# Autodesk Inventor assembly: ShfiterAssy
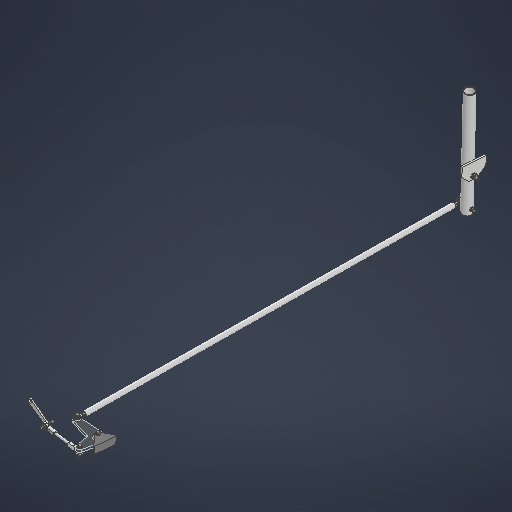
[picture p0: Inventor's stored thumbnail of the model, 512x512]
Saved by Autodesk Inventor 2026.2 (Build 302298010, 298A)
## iProperties
Created: 2026-07-07
Part Number: ShfiterAssy
Document SubType Name: Assembly
Designer: tasle
Author: tasle
## Documents named in this file (18)
- C:\Users\tasle\Documents\PersonalProjects\FSAE\GOGO_FSAE_CAD\Shifter\ShfiterAssy.iam
- C:\Users\tasle\Documents\PersonalProjects\FSAE\GOGO_FSAE_CAD\Shifter\crank.ipt
- C:\Users\tasle\Documents\PersonalProjects\FSAE\GOGO_FSAE_CAD\Shifter\59935K71_Ball Joint Rod End\59935K71_Ball Joint Rod End\59935K71_Ball Joint Rod End.ipt
- C:\Users\tasle\Documents\PersonalProjects\FSAE\GOGO_FSAE_CAD\Shifter\threadedtubeshort.ipt
- C:\Users\tasle\Documents\Inventor\Content Center Files\R2026\en-US\ISO 4162\ISO 4162 - M5 x 25.ipt
- C:\Users\tasle\Documents\Inventor\Content Center Files\R2026\en-US\ISO 4161\ISO 4161 - M5(1).ipt
- C:\Users\tasle\Documents\PersonalProjects\FSAE\GOGO_FSAE_CAD\Shifter\ShifterBracket.ipt
- C:\Users\tasle\Documents\PersonalProjects\FSAE\GOGO_FSAE_CAD\Shifter\BellCrank.ipt
- C:\Users\tasle\Documents\PersonalProjects\FSAE\GOGO_FSAE_CAD\Shifter\Bearing.ipt
- C:\Users\tasle\Documents\PersonalProjects\FSAE\GOGO_FSAE_CAD\Shifter\spacer.ipt
- C:\Users\tasle\Documents\PersonalProjects\FSAE\GOGO_FSAE_CAD\Shifter\6045N121_Low-Carbon Steel Round Tube\6045N121_Low-Carbon Steel Round Tube\6045N121_Low-Carbon Steel Round Tube.ipt
- C:\Users\tasle\Documents\PersonalProjects\FSAE\GOGO_FSAE_CAD\Shifter\59935K81_Ball Joint Rod End\59935K81_Ball Joint Rod End\59935K81_Ball Joint Rod End.ipt
- C:\Users\tasle\Documents\Inventor\Content Center Files\R2026\en-US\ISO 4032(2)\ISO 4032 - M5 - ISO.ipt
- C:\Users\tasle\Documents\PersonalProjects\FSAE\GOGO_FSAE_CAD\Shifter\stickplate.ipt
- C:\Users\tasle\Documents\PersonalProjects\FSAE\GOGO_FSAE_CAD\Shifter\stickshift.ipt
- C:\Users\tasle\Documents\Inventor\Content Center Files\R2026\en-US\ISO 4162\ISO 4162 - M5 x 45.ipt
- C:\Users\tasle\Documents\Inventor\Content Center Files\R2026\en-US\ISO 4162\ISO 4162 - M6 x 40.ipt
- C:\Users\tasle\Documents\Inventor\Content Center Files\R2026\en-US\ISO 4161\ISO 4161 - M6(1).ipt
## Components (28 placed, 17 different names)
1. crank:1 — Rotational:1, Rotational:5
2. 59935K71_Ball Joint Rod End:1 — Rotational:1, Rotational:2, Rotational:4
3. 59935K71_Ball Joint Rod End:2 — Rotational:3, Rotational:10, Rotational:12
4. threadedtubeshort:1 — Rotational:2, Rotational:3
5. ISO 4162 M5 x 25:1 — Rotational:4
6. ISO 4162 M5 x 25:2 — Rotational:11
7. ISO 4161 M5:1 — Rotational:5
8. ISO 4161 M5:3 — Rotational:12
9. ShifterBracket:1 — Rotational:9, Rotational:18, Rotational:19
10. BellCrank:1 — Rotational:6, Rotational:10, Rotational:11, Rotational:15, Rotational:17
11. Bearing:1 — Rotational:6, Rotational:7, Rotational:8
12. spacer:1 — Rotational:8
13. spacer:2 — Rotational:7, Rotational:9
14. 6045N121_Low-Carbon Steel Round Tube:1 — Rigid:1, Rigid:2
15. 59935K81_Ball Joint Rod End:1 — Rotational:14, Rotational:15, Rotational:16
16. 59935K81_Ball Joint Rod End:2 — Rotational:13, Rotational:21, Rotational:23
17. ISO 4032 M5:1 — Rigid:1, Rotational:14
18. ISO 4032 M5:2 — Rigid:2, Rotational:13
19. ISO 4162 M5 x 25:3 — Rotational:16
20. ISO 4161 M5:4 — Rotational:17
21. ISO 4162 M5 x 25:4 — Rotational:18
22. ISO 4161 M5:5 — Rotational:19
23. stickplate:1 — Rotational:20, Rotational:22
24. stickshift:1 — Rotational:20, Rotational:21, Rigid:3, Rigid:4
25. ISO 4162 M5 x 45:1 — Rotational:23
26. ISO 4162 M6 x 40:1 — Rigid:3
27. ISO 4161 M5:6 — Rigid:4
28. ISO 4161 M6:1 — Rotational:22
## Relationships (27: RevoluteJoint 23, WeldJoint 4)
- Rotational:1 [RevoluteJoint]: crank:1 ↔ 59935K71_Ball Joint Rod End:1
- Rotational:2 [RevoluteJoint]: 59935K71_Ball Joint Rod End:1 ↔ threadedtubeshort:1
- Rotational:3 [RevoluteJoint]: 59935K71_Ball Joint Rod End:2 ↔ threadedtubeshort:1
- Rotational:4 [RevoluteJoint]: 59935K71_Ball Joint Rod End:1 ↔ ISO 4162 M5 x 25:1
- Rotational:5 [RevoluteJoint]: crank:1 ↔ ISO 4161 M5:1
- Rotational:6 [RevoluteJoint]: BellCrank:1 ↔ Bearing:1
- Rotational:7 [RevoluteJoint]: Bearing:1 ↔ spacer:2
- Rotational:8 [RevoluteJoint]: Bearing:1 ↔ spacer:1
- Rotational:9 [RevoluteJoint]: ShifterBracket:1 ↔ spacer:2
- Rotational:10 [RevoluteJoint]: 59935K71_Ball Joint Rod End:2 ↔ BellCrank:1
- Rotational:11 [RevoluteJoint]: ISO 4162 M5 x 25:2 ↔ BellCrank:1
- Rotational:12 [RevoluteJoint]: 59935K71_Ball Joint Rod End:2 ↔ ISO 4161 M5:3
- Rigid:1 [WeldJoint]: 6045N121_Low-Carbon Steel Round Tube:1 ↔ ISO 4032 M5:1
- Rigid:2 [WeldJoint]: 6045N121_Low-Carbon Steel Round Tube:1 ↔ ISO 4032 M5:2
- Rotational:13 [RevoluteJoint]: 59935K81_Ball Joint Rod End:2 ↔ ISO 4032 M5:2
- Rotational:14 [RevoluteJoint]: 59935K81_Ball Joint Rod End:1 ↔ ISO 4032 M5:1
- Rotational:15 [RevoluteJoint]: BellCrank:1 ↔ 59935K81_Ball Joint Rod End:1
- Rotational:16 [RevoluteJoint]: 59935K81_Ball Joint Rod End:1 ↔ ISO 4162 M5 x 25:3
- Rotational:17 [RevoluteJoint]: BellCrank:1 ↔ ISO 4161 M5:4
- Rotational:18 [RevoluteJoint]: ShifterBracket:1 ↔ ISO 4162 M5 x 25:4
- Rotational:19 [RevoluteJoint]: ShifterBracket:1 ↔ ISO 4161 M5:5
- Rotational:20 [RevoluteJoint]: stickplate:1 ↔ stickshift:1
- Rotational:21 [RevoluteJoint]: 59935K81_Ball Joint Rod End:2 ↔ stickshift:1
- Rigid:3 [WeldJoint]: stickshift:1 ↔ ISO 4162 M6 x 40:1
- Rotational:22 [RevoluteJoint]: stickplate:1 ↔ ISO 4161 M6:1
- Rotational:23 [RevoluteJoint]: 59935K81_Ball Joint Rod End:2 ↔ ISO 4162 M5 x 45:1
- Rigid:4 [WeldJoint] (-2 mm): stickshift:1 ↔ ISO 4161 M5:6
